# Autodesk Inventor assembly: right_Arm
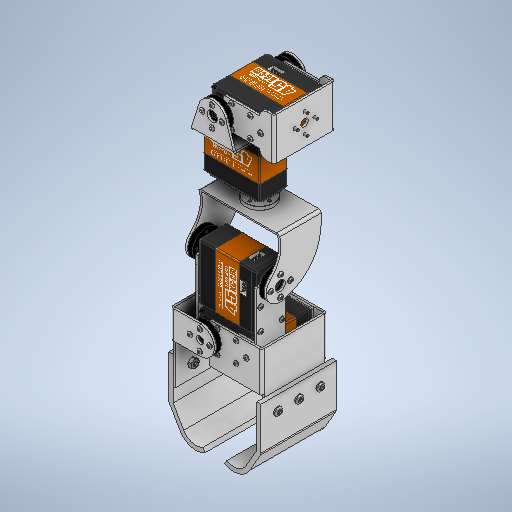
[picture p0: Inventor's stored thumbnail of the model, 512x512]
Saved by Autodesk Inventor 2026.1 (Build 301233000, 233)
## iProperties
Created: 2025-07-28
Part Number: right_Arm
Document SubType Name: Assembly
Designer: LG
Author: LG
## Documents named in this file (19)
- C:\Users\chris\Documents\Inventor\RHp_Humanoid_ver1\Total\right_Arm.iam
- C:\Users\chris\Documents\Inventor\RHp_Humanoid_ver1\Part_Arm\HTD-45H, Horn\HTD-45H\HTD-45H.iam
- C:\Users\chris\Documents\Inventor\RHp_Humanoid_ver1\Part_Arm\HTD-45H, Horn\Horn\Top Horn.ipt
- C:\Users\chris\Documents\Inventor\RHp_Humanoid_ver1\Part_Arm\Frame\Arm\axis_18_top_frame.ipt
- C:\Users\chris\Documents\Inventor\RHp_Humanoid_ver1\Part_Arm\HTD-45H, Horn\Horn\Bottom Horn.ipt
- C:\Users\chris\Documents\Inventor\RHp_Humanoid_ver1\Part_Arm\Frame\Arm\axis_19_bottom_frame.ipt
- C:\Users\chris\Documents\Inventor\RHp_Humanoid_ver1\Part_Arm\Frame\Arm\axis_20_bottom_frame.ipt
- C:\Users\chris\Documents\Inventor\RHp_Humanoid_ver1\Part_Arm\Frame\Arm\axis_21_top_frame.ipt
- C:\Users\chris\Documents\Inventor\RHp_Humanoid_ver1\Part_Arm\Frame\Arm\axis_21_bottom_frame.ipt
- C:\Users\chris\Documents\Inventor\RHp_Humanoid_ver1\Part_Arm\Frame\Arm\axis_22_bottom_frame.ipt
- C:\Users\chris\Documents\Inventor\RHp_Humanoid_ver1\Part_Arm\Frame\Arm\axis_22_top_frame.ipt
- C:\Users\chris\Documents\Inventor\RHp_Humanoid_ver1\Part_Arm\Frame\Arm\HTD-45H_no bottom horn.ipt
- C:\Users\chris\Documents\Inventor\RHp_Humanoid_ver1\Part_Arm\Frame\Arm\gripper_frame.ipt
- C:\Users\chris\Documents\Inventor\RHp_Humanoid_ver1\Part_Arm\Bolt, Bearing, Nut, Washer\볼트, 너트\M2x4 Bolt.ipt
- C:\Users\chris\Documents\Inventor\RHp_Humanoid_ver1\Part_Arm\Bolt, Bearing, Nut, Washer\볼트, 너트\M3x6 Bolt.ipt
- C:\Users\chris\Documents\Inventor\RHp_Humanoid_ver1\Part_Arm\Bolt, Bearing, Nut, Washer\볼트, 너트\M3 Nut.ipt
- C:\Users\chris\Documents\Inventor\RHp_Humanoid_ver1\Part_Arm\Bolt, Bearing, Nut, Washer\볼트, 너트\M2x6 Bolt.ipt
- C:\Users\chris\Documents\Inventor\RHp_Humanoid_ver1\Part_Arm\Bolt, Bearing, Nut, Washer\볼트, 너트\M3x8 Bolt.ipt
- C:\Users\chris\Documents\Inventor\RHp_Humanoid_ver1\Part_Arm\HTD-45H, Horn\Horn\Top Horn silver.ipt
## Components (103 placed, 17 different names)
1. M2x4 Bolt:67 — Rigid:116
2. M2x4 Bolt:66 — Rigid:114
3. M2x4 Bolt:65 — Rigid:115
4. M2x4 Bolt:64 — Rigid:113
5. M2x4 Bolt:63 — Rigid:112
6. M2x4 Bolt:62 — Rigid:110
7. M2x4 Bolt:61 — Rigid:109
8. M2x4 Bolt:60 — Rigid:111
9. M2x4 Bolt:59 — Rigid:108
10. M2x4 Bolt:21 — Rigid:22
11. M2x4 Bolt:20 — Rigid:21
12. M2x4 Bolt:19 — Rigid:20
13. M2x4 Bolt:18 — Rigid:19
14. axis_18_top_frame:1 — Mate:7, Mate:8, Mate:9, Rigid:19, Rigid:20, Rigid:21, Rigid:22, Rigid:108, Rigid:109, Rigid:110, Rigid:111, Rigid:112, Rigid:113, Rigid:114, Rigid:115, Rigid:116
15. M2x4 Bolt:2 — Rigid:7
16. M2x4 Bolt:4 — Rigid:9
17. M2x4 Bolt:5 — Rigid:8
18. M2x4 Bolt:3 — Rigid:10
19. M2x4 Bolt:13 — Rigid:15
20. M2x4 Bolt:12 — Rigid:17
21. M2x4 Bolt:15 — Rigid:18
22. M2x4 Bolt:14 — Rigid:16
23. M2x4 Bolt:55 — Rigid:96
24. M2x4 Bolt:56 — Rigid:98
25. M2x4 Bolt:57 — Rigid:95
26. M2x4 Bolt:58 — Rigid:97
27. axis_19_bottom_frame:1 — Flush:2, Mate:12, Mate:13, Rigid:7, Rigid:8, Rigid:9, Rigid:10, Rigid:15, Rigid:16, Rigid:17, Rigid:18, Mate:49, Mate:50, Flush:15, Rigid:95, Rigid:96, Rigid:97, Rigid:98
28. Bottom Horn:1 — Mate:10, Mate:11, Flush:1
29. Top Horn:2 — Rotational:2, Flush:2, Mate:12, Mate:13
30. HTD-45H:2 [sub-assembly] — Mate:7, Mate:8, Mate:9, Rotational:2, Mate:10, Mate:11, Flush:1
31. M2x4 Bolt:27 — Rigid:27
32. M2x4 Bolt:28 — Rigid:29
33. M2x4 Bolt:29 — Rigid:30
34. M2x4 Bolt:26 — Rigid:28
35. axis_20_bottom_frame:1 — Mate:29, Mate:30, Mate:31, Rigid:27, Rigid:28, Rigid:29, Rigid:30, Rigid:31, Rigid:32, Rigid:33, Rigid:34, Rigid:35, Rigid:36, Rigid:37, Rigid:38, Mate:51, Mate:52, Flush:16
36. Top Horn silver:2 — Rotational:3, Mate:51, Mate:52, Flush:16
37. HTD-45H:6 — Mate:49, Mate:50, Flush:15, Rotational:3
38. M2x4 Bolt:30 — Rigid:31
39. M2x4 Bolt:31 — Rigid:32
40. M2x4 Bolt:33 — Rigid:33
41. M2x4 Bolt:32 — Rigid:34
42. M2x4 Bolt:34 — Rigid:35
43. M2x4 Bolt:35 — Rigid:37
44. M2x4 Bolt:36 — Rigid:36
45. M2x4 Bolt:37 — Rigid:38
46. M2x4 Bolt:43 — Rigid:44
47. M2x4 Bolt:44 — Rigid:45
48. M2x4 Bolt:45 — Rigid:46
49. M2x4 Bolt:46 — Rigid:47
50. M2x4 Bolt:39 — Rigid:40
51. M2x4 Bolt:38 — Rigid:39
52. M2x4 Bolt:41 — Rigid:42
53. M2x4 Bolt:40 — Rigid:41
54. M2x4 Bolt:42 — Rigid:43
55. M3 Nut:3 — Rigid:64
56. M3 Nut:4 — Rigid:62
57. M3 Nut:2 — Rigid:63
58. M3 Nut:1 — Rigid:61
59. M3x6 Bolt:1 — Rigid:58
60. M3x6 Bolt:2 — Rigid:59
61. M3x6 Bolt:3 — Rigid:60
62. M3x6 Bolt:4 — Rigid:57
63. axis_21_top_frame:1 — Mate:36, Mate:37, Mate:38, Mate:39, Mate:45, Rigid:39, Rigid:40, Rigid:41, Rigid:42, Rigid:43, Rigid:44, Rigid:45, Rigid:46, Rigid:47, Rigid:57, Rigid:58, Rigid:59, Rigid:60
64. axis_21_bottom_frame:1 — Mate:39, Mate:40, Flush:10, Mate:44, Flush:11, Rigid:61, Rigid:62, Rigid:63, Rigid:64
65. Bottom Horn:2 — Mate:27, Flush:7, Mate:28
66. Top Horn:4 — Rotational:4, Mate:29, Mate:30, Mate:31
67. HTD-45H:4 [sub-assembly] — Mate:27, Flush:7, Mate:28, Rotational:4, Mate:35, Flush:8, Flush:9, Mate:37, Mate:38
68. M2x6 Bolt:1 — Rigid:99
69. M2x6 Bolt:2 — Rigid:103
70. M2x6 Bolt:3 — Rigid:100
71. M2x6 Bolt:4 — Rigid:102
72. M2x6 Bolt:5 — Rigid:101
73. M2x6 Bolt:6 — Rigid:104
74. M2x6 Bolt:7 — Rigid:105
75. M2x6 Bolt:8 — Rigid:107
76. M2x6 Bolt:9 — Rigid:106
77. M2x4 Bolt:47 — Rigid:65
78. M2x4 Bolt:49 — Rigid:66
79. M2x4 Bolt:50 — Rigid:68
80. M2x4 Bolt:48 — Rigid:67
81. M2x4 Bolt:54 — Rigid:69
82. M2x4 Bolt:51 — Rigid:70
83. M2x4 Bolt:53 — Rigid:72
84. M2x4 Bolt:52 — Rigid:71
85. M3x8 Bolt:4 — Rigid:88
86. M3x8 Bolt:5 — Rigid:89
87. M3x8 Bolt:6 — Rigid:90
88. M3 Nut:10 — Rigid:93
89. M3 Nut:9 — Rigid:92
90. M3 Nut:8 — Rigid:91
91. M3x8 Bolt:3 — Rigid:84
92. M3x8 Bolt:2 — Rigid:83
93. M3x8 Bolt:1 — Rigid:82
94. M3 Nut:6 — Rigid:87
95. M3 Nut:7 — Rigid:86
96. M3 Nut:5 — Rigid:85
97. axis_22_bottom_frame:1 — Mate:41, Mate:42, Mate:43, Rigid:1, Rigid:65, Rigid:66, Rigid:67, Rigid:68, Rigid:69, Rigid:70, Rigid:71, Rigid:72, Rigid:85, Rigid:86, Rigid:87
98. axis_22_top_frame:1 — Mate:44, Flush:11, Mate:45, Rigid:91, Rigid:92, Rigid:93, Rigid:94, Rigid:99, Rigid:100, Rigid:101, Rigid:102, Rigid:103, Rigid:104, Rigid:105, Rigid:106, Rigid:107
99. gripper_frame:1 — Rigid:1, Rigid:82, Rigid:83, Rigid:84
100. gripper_frame:2 — Rigid:88, Rigid:89, Rigid:90, Rigid:94
101. Top Horn:5 — Rotational:5, Mate:41, Mate:42, Mate:43
102. Bottom Horn:3 — Mate:32, Mate:33, Mate:34
103. HTD-45H:5 [sub-assembly] — Rotational:5, Mate:32, Mate:33, Mate:34, Mate:35, Flush:8, Flush:9, Mate:36, Mate:40, Flush:10
## Relationships (128: WeldJoint 85, Mate 30, Flush 9, RevoluteJoint 4)
- Rotational:2 [RevoluteJoint]: Top Horn:2 ↔ HTD-45H:2
- Rotational:3 [RevoluteJoint]: Top Horn silver:2 ↔ HTD-45H:6
- Rotational:4 [RevoluteJoint]: Top Horn:4 ↔ HTD-45H:4
- Rotational:5 [RevoluteJoint]: Top Horn:5 ↔ HTD-45H:5
- Mate:7: axis_18_top_frame:1 ↔ HTD-45H:2
- Mate:8 (5 mm): axis_18_top_frame:1 ↔ HTD-45H:2
- Mate:9: axis_18_top_frame:1 ↔ HTD-45H:2
- Mate:10: Bottom Horn:1 ↔ HTD-45H:2
- Mate:11: Bottom Horn:1 ↔ HTD-45H:2
- Flush:1: Bottom Horn:1 ↔ HTD-45H:2
- Flush:2 (14.5 mm): axis_19_bottom_frame:1 ↔ Top Horn:2
- Mate:12: axis_19_bottom_frame:1 ↔ Top Horn:2
- Mate:13: axis_19_bottom_frame:1 ↔ Top Horn:2
- Mate:27: Bottom Horn:2 ↔ HTD-45H:4
- Flush:7: Bottom Horn:2 ↔ HTD-45H:4
- Mate:28: Bottom Horn:2 ↔ HTD-45H:4
- Mate:29 (30.43 mm): axis_20_bottom_frame:1 ↔ Top Horn:4
- Mate:30 (-14 mm): axis_20_bottom_frame:1 ↔ Top Horn:4
- Mate:31: axis_20_bottom_frame:1 ↔ Top Horn:4
- Mate:32: Bottom Horn:3 ↔ HTD-45H:5
- Mate:33: Bottom Horn:3 ↔ HTD-45H:5
- Mate:34: Bottom Horn:3 ↔ HTD-45H:5
- Mate:35 (3 mm): HTD-45H:4 ↔ HTD-45H:5
- Flush:8: HTD-45H:4 ↔ HTD-45H:5
- Flush:9: HTD-45H:4 ↔ HTD-45H:5
- Mate:36 (5 mm): axis_21_top_frame:1 ↔ HTD-45H:5
- Mate:37: axis_21_top_frame:1 ↔ HTD-45H:4
- Mate:38: axis_21_top_frame:1 ↔ HTD-45H:4
- Mate:39: axis_21_top_frame:1 ↔ axis_21_bottom_frame:1
- Mate:40: axis_21_bottom_frame:1 ↔ HTD-45H:5
- Flush:10: axis_21_bottom_frame:1 ↔ HTD-45H:5
- Mate:41: axis_22_bottom_frame:1 ↔ Top Horn:5
- Mate:42: axis_22_bottom_frame:1 ↔ Top Horn:5
- Mate:43 (19.43 mm): axis_22_bottom_frame:1 ↔ Top Horn:5
- Mate:44: axis_21_bottom_frame:1 ↔ axis_22_top_frame:1
- Flush:11: axis_21_bottom_frame:1 ↔ axis_22_top_frame:1
- Mate:45 (5 mm): axis_21_top_frame:1 ↔ axis_22_top_frame:1
- Rigid:1 [WeldJoint]: axis_22_bottom_frame:1 ↔ gripper_frame:1
- Rigid:7 [WeldJoint]: M2x4 Bolt:2 ↔ axis_19_bottom_frame:1
- Rigid:8 [WeldJoint]: M2x4 Bolt:5 ↔ axis_19_bottom_frame:1
- Rigid:9 [WeldJoint]: M2x4 Bolt:4 ↔ axis_19_bottom_frame:1
- Rigid:10 [WeldJoint]: M2x4 Bolt:3 ↔ axis_19_bottom_frame:1
- Rigid:15 [WeldJoint]: M2x4 Bolt:13 ↔ axis_19_bottom_frame:1
- Rigid:16 [WeldJoint]: M2x4 Bolt:14 ↔ axis_19_bottom_frame:1
- Rigid:17 [WeldJoint]: M2x4 Bolt:12 ↔ axis_19_bottom_frame:1
- Rigid:18 [WeldJoint]: M2x4 Bolt:15 ↔ axis_19_bottom_frame:1
- Rigid:19 [WeldJoint]: M2x4 Bolt:18 ↔ axis_18_top_frame:1
- Rigid:20 [WeldJoint]: M2x4 Bolt:19 ↔ axis_18_top_frame:1
- Rigid:21 [WeldJoint]: M2x4 Bolt:20 ↔ axis_18_top_frame:1
- Rigid:22 [WeldJoint]: M2x4 Bolt:21 ↔ axis_18_top_frame:1
- Rigid:27 [WeldJoint]: M2x4 Bolt:27 ↔ axis_20_bottom_frame:1
- Rigid:28 [WeldJoint]: M2x4 Bolt:26 ↔ axis_20_bottom_frame:1
- Rigid:29 [WeldJoint]: M2x4 Bolt:28 ↔ axis_20_bottom_frame:1
- Rigid:30 [WeldJoint]: M2x4 Bolt:29 ↔ axis_20_bottom_frame:1
- Rigid:31 [WeldJoint]: axis_20_bottom_frame:1 ↔ M2x4 Bolt:30
- Rigid:32 [WeldJoint]: axis_20_bottom_frame:1 ↔ M2x4 Bolt:31
- Rigid:33 [WeldJoint]: axis_20_bottom_frame:1 ↔ M2x4 Bolt:33
- Rigid:34 [WeldJoint]: axis_20_bottom_frame:1 ↔ M2x4 Bolt:32
- Rigid:35 [WeldJoint]: axis_20_bottom_frame:1 ↔ M2x4 Bolt:34
- Rigid:36 [WeldJoint]: axis_20_bottom_frame:1 ↔ M2x4 Bolt:36
- Rigid:37 [WeldJoint]: axis_20_bottom_frame:1 ↔ M2x4 Bolt:35
- Rigid:38 [WeldJoint]: axis_20_bottom_frame:1 ↔ M2x4 Bolt:37
- Rigid:39 [WeldJoint]: M2x4 Bolt:38 ↔ axis_21_top_frame:1
- Rigid:40 [WeldJoint]: M2x4 Bolt:39 ↔ axis_21_top_frame:1
- Rigid:41 [WeldJoint]: M2x4 Bolt:40 ↔ axis_21_top_frame:1
- Rigid:42 [WeldJoint]: M2x4 Bolt:41 ↔ axis_21_top_frame:1
- Rigid:43 [WeldJoint]: M2x4 Bolt:42 ↔ axis_21_top_frame:1
- Rigid:44 [WeldJoint]: M2x4 Bolt:43 ↔ axis_21_top_frame:1
- Rigid:45 [WeldJoint]: M2x4 Bolt:44 ↔ axis_21_top_frame:1
- Rigid:46 [WeldJoint]: M2x4 Bolt:45 ↔ axis_21_top_frame:1
- Rigid:47 [WeldJoint]: M2x4 Bolt:46 ↔ axis_21_top_frame:1
- Rigid:57 [WeldJoint]: M3x6 Bolt:4 ↔ axis_21_top_frame:1
- Rigid:58 [WeldJoint]: M3x6 Bolt:1 ↔ axis_21_top_frame:1
- Rigid:59 [WeldJoint]: M3x6 Bolt:2 ↔ axis_21_top_frame:1
- Rigid:60 [WeldJoint]: M3x6 Bolt:3 ↔ axis_21_top_frame:1
- Rigid:61 [WeldJoint]: M3 Nut:1 ↔ axis_21_bottom_frame:1
- Rigid:62 [WeldJoint]: M3 Nut:4 ↔ axis_21_bottom_frame:1
- Rigid:63 [WeldJoint]: M3 Nut:2 ↔ axis_21_bottom_frame:1
- Rigid:64 [WeldJoint]: M3 Nut:3 ↔ axis_21_bottom_frame:1
- Rigid:65 [WeldJoint]: M2x4 Bolt:47 ↔ axis_22_bottom_frame:1
- Rigid:66 [WeldJoint]: M2x4 Bolt:49 ↔ axis_22_bottom_frame:1
- Rigid:67 [WeldJoint]: M2x4 Bolt:48 ↔ axis_22_bottom_frame:1
- Rigid:68 [WeldJoint]: M2x4 Bolt:50 ↔ axis_22_bottom_frame:1
- Rigid:69 [WeldJoint]: M2x4 Bolt:54 ↔ axis_22_bottom_frame:1
- Rigid:70 [WeldJoint]: M2x4 Bolt:51 ↔ axis_22_bottom_frame:1
- Rigid:71 [WeldJoint]: M2x4 Bolt:52 ↔ axis_22_bottom_frame:1
- Rigid:72 [WeldJoint]: M2x4 Bolt:53 ↔ axis_22_bottom_frame:1
- Rigid:82 [WeldJoint]: M3x8 Bolt:1 ↔ gripper_frame:1
- Rigid:83 [WeldJoint]: M3x8 Bolt:2 ↔ gripper_frame:1
- Rigid:84 [WeldJoint]: M3x8 Bolt:3 ↔ gripper_frame:1
- Rigid:85 [WeldJoint]: M3 Nut:5 ↔ axis_22_bottom_frame:1
- Rigid:86 [WeldJoint]: M3 Nut:7 ↔ axis_22_bottom_frame:1
- Rigid:87 [WeldJoint]: M3 Nut:6 ↔ axis_22_bottom_frame:1
- Rigid:88 [WeldJoint]: M3x8 Bolt:4 ↔ gripper_frame:2
- Rigid:89 [WeldJoint]: M3x8 Bolt:5 ↔ gripper_frame:2
- Rigid:90 [WeldJoint]: M3x8 Bolt:6 ↔ gripper_frame:2
- Rigid:91 [WeldJoint]: M3 Nut:8 ↔ axis_22_top_frame:1
- Rigid:92 [WeldJoint]: M3 Nut:9 ↔ axis_22_top_frame:1
- Rigid:93 [WeldJoint]: M3 Nut:10 ↔ axis_22_top_frame:1
- Rigid:94 [WeldJoint]: axis_22_top_frame:1 ↔ gripper_frame:2
- Mate:49: axis_19_bottom_frame:1 ↔ HTD-45H:6
- Mate:50: axis_19_bottom_frame:1 ↔ HTD-45H:6
- Flush:15: axis_19_bottom_frame:1 ↔ HTD-45H:6
- Rigid:95 [WeldJoint]: M2x4 Bolt:57 ↔ axis_19_bottom_frame:1
- Rigid:96 [WeldJoint]: M2x4 Bolt:55 ↔ axis_19_bottom_frame:1
- Rigid:97 [WeldJoint]: M2x4 Bolt:58 ↔ axis_19_bottom_frame:1
- Rigid:98 [WeldJoint]: M2x4 Bolt:56 ↔ axis_19_bottom_frame:1
- Rigid:99 [WeldJoint]: M2x6 Bolt:1 ↔ axis_22_top_frame:1
- Rigid:100 [WeldJoint]: M2x6 Bolt:3 ↔ axis_22_top_frame:1
- Rigid:101 [WeldJoint]: M2x6 Bolt:5 ↔ axis_22_top_frame:1
- Rigid:102 [WeldJoint]: M2x6 Bolt:4 ↔ axis_22_top_frame:1
- Rigid:103 [WeldJoint]: M2x6 Bolt:2 ↔ axis_22_top_frame:1
- Rigid:104 [WeldJoint]: M2x6 Bolt:6 ↔ axis_22_top_frame:1
- Rigid:105 [WeldJoint]: M2x6 Bolt:7 ↔ axis_22_top_frame:1
- Rigid:106 [WeldJoint]: M2x6 Bolt:9 ↔ axis_22_top_frame:1
- Rigid:107 [WeldJoint]: M2x6 Bolt:8 ↔ axis_22_top_frame:1
- Rigid:108 [WeldJoint]: M2x4 Bolt:59 ↔ axis_18_top_frame:1
- Rigid:109 [WeldJoint]: M2x4 Bolt:61 ↔ axis_18_top_frame:1
- Rigid:110 [WeldJoint]: M2x4 Bolt:62 ↔ axis_18_top_frame:1
- Rigid:111 [WeldJoint]: M2x4 Bolt:60 ↔ axis_18_top_frame:1
- Rigid:112 [WeldJoint]: M2x4 Bolt:63 ↔ axis_18_top_frame:1
- Rigid:113 [WeldJoint]: M2x4 Bolt:64 ↔ axis_18_top_frame:1
- Rigid:114 [WeldJoint]: M2x4 Bolt:66 ↔ axis_18_top_frame:1
- Rigid:115 [WeldJoint]: M2x4 Bolt:65 ↔ axis_18_top_frame:1
- Rigid:116 [WeldJoint]: M2x4 Bolt:67 ↔ axis_18_top_frame:1
- Mate:51: axis_20_bottom_frame:1 ↔ Top Horn silver:2
- Mate:52: axis_20_bottom_frame:1 ↔ Top Horn silver:2
- Flush:16: axis_20_bottom_frame:1 ↔ Top Horn silver:2
